# Autodesk Inventor assembly: shuttle-carrier-nn32
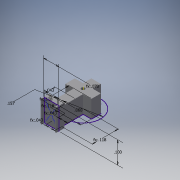
[picture p0: Inventor's stored thumbnail of the model, 180x180]
Saved by Autodesk Inventor 2016 (Build 200138000, 138)
## iProperties
Created: 2016-07-02
Part Number: shuttle-carrier-nn32
Document SubType Name: Assembly
Designer: GentnerLab
Author: GentnerLab
## Documents named in this file (3)
- C:\Users\GentnerLab\Documents\Inventor\Parts\new_drive\60unm-6mm\shuttle-carrier-nn32.iam
- C:\Users\GentnerLab\Documents\GentnerLabSTL\probe_carrier_nn32.ipt
- C:\Users\GentnerLab\Documents\Inventor\Parts\new_drive\60unm-6mm\shuttle.ipt
## Components (2 placed, 2 different names)
1. probe_carrier_nn32:1 — Mate:1, Mate:2
2. shuttle:1 — Mate:1, Mate:2
## Relationships (2: Mate 2)
- Mate:1 (0.3683 mm): probe_carrier_nn32:1 ↔ shuttle:1
- Mate:2: probe_carrier_nn32:1 ↔ shuttle:1
